# Autodesk Inventor assembly: Assembly9
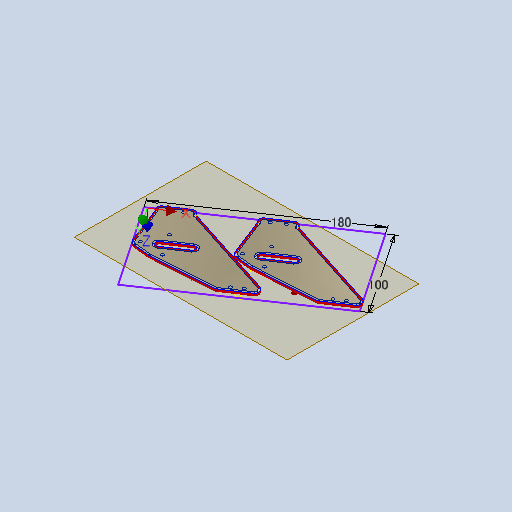
[picture p0: Inventor's stored thumbnail of the model, 512x512]
Saved by Autodesk Inventor 2025.2 (Build 292293000, 293)
## iProperties
Created: 2024-12-26
Part Number: Assembly9
Document SubType Name: Assembly
Designer: haruy
Author: haruy
## Documents named in this file (2)
- C:\Users\haruy\Documents\ロボコン\NHK2025\cad\cnc\Assembly9.iam
- C:\Users\haruy\Documents\ロボコン\NHK2025\cad\nagahisa\belt_liner\belt_liner_v1_Plate_8.ipt
## Components (2 placed, 1 different names)
1. belt_liner_v1_Plate_8:1 — フラッシュ:1, フラッシュ:3
2. belt_liner_v1_Plate_8:2 — フラッシュ:2, フラッシュ:3
## Relationships (3: Flush 3)
- フラッシュ:1 [Flush]: belt_liner_v1_Plate_8:1
- フラッシュ:2 [Flush]: belt_liner_v1_Plate_8:2
- フラッシュ:3 [Flush]: belt_liner_v1_Plate_8:1 ↔ belt_liner_v1_Plate_8:2
